# Autodesk Inventor assembly: LegAssembly
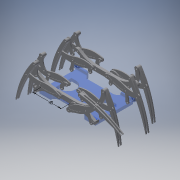
[picture p0: Inventor's stored thumbnail of the model, 180x180]
Saved by Autodesk Inventor 2017.2 (Build 212233000, 233)
## iProperties
Created: 2016-08-27
Part Number: LegAssembly
Document SubType Name: Assembly
Designer: Nic
Author: Nic
## Documents named in this file (8)
- C:\Users\Nic\Documents\TermiteBeest\LegAssembly.iam
- C:\Users\Nic\Documents\TermiteBeest\legFrame.ipt
- C:\Users\Nic\Documents\TermiteBeest\linkageC.ipt
- C:\Users\Nic\Documents\TermiteBeest\legB.ipt
- C:\Users\Nic\Documents\TermiteBeest\linkageB.ipt
- C:\Users\Nic\Documents\TermiteBeest\legA.ipt
- C:\Users\Nic\Documents\TermiteBeest\linkageA.ipt
- C:\Users\Nic\Documents\TermiteBeest\baseplate.ipt
## Components (43 placed, 7 different names)
1. legFrame:1 — Insert:1, Insert:3, Insert:4, Insert:5, Insert:6, Insert:7, Insert:8, Insert:9, Insert:10, Insert:11, Insert:12, Insert:13, Insert:14, Insert:15, Insert:61
2. legB:1 — Insert:16, Insert:17, Insert:18
3. linkageB:1 — Insert:3, Insert:4, Insert:16
4. legA:1 — Insert:17, Insert:19
5. linkageA:1 — Insert:5, Insert:19
6. linkageC:1 — Insert:6, Insert:18
7. linkageC:2 — Insert:8, Insert:20
8. linkageB:2 — Insert:7, Insert:21
9. linkageA:2 — Insert:9, Insert:22
10. legB:2 — Insert:20, Insert:21, Insert:23
11. legA:2 — Insert:22, Insert:23
12. linkageC:3 — Insert:10, Insert:24
13. linkageA:3 — Insert:11, Insert:25
14. linkageB:3 — Insert:12, Insert:26
15. legA:3 — Insert:25, Insert:27
16. legB:3 — Insert:24, Insert:26, Insert:27
17. linkageB:4 — Insert:13, Insert:28
18. linkageA:4 — Insert:15, Insert:29
19. linkageC:4 — Insert:14, Insert:30
20. legA:4 — Insert:29, Insert:31
21. legB:4 — Insert:28, Insert:30, Insert:31
22. baseplate:1 — Insert:1, Insert:32, Insert:61, Insert:62
23. linkageC:5 — Insert:34, Insert:35
24. linkageC:6 — Insert:36, Insert:37
25. legFrame:2 — Insert:32, Insert:33, Insert:34, Insert:36, Insert:38, Insert:39, Insert:40, Insert:41, Insert:42, Insert:43, Insert:44, Insert:45, Insert:53, Insert:62
26. linkageA:6 — Insert:38, Insert:46
27. linkageA:7 — Insert:39, Insert:47
28. legA:5 — Insert:47, Insert:48
29. legA:6 — Insert:46, Insert:49
30. legB:5 — Insert:35, Insert:48, Insert:50
31. legB:6 — Insert:37, Insert:49, Insert:51
32. linkageB:5 — Insert:40, Insert:50
33. linkageB:6 — Insert:41, Insert:51
34. linkageC:7 — Insert:42, Insert:52
35. linkageC:8 — Insert:53, Insert:54
36. linkageB:7 — Insert:33, Insert:55
37. linkageB:8 — Insert:45, Insert:56
38. linkageA:8 — Insert:43, Insert:57
39. linkageA:9 — Insert:44, Insert:58
40. legA:7 — Insert:57, Insert:59
41. legA:8 — Insert:58, Insert:60
42. legB:7 — Insert:54, Insert:55, Insert:59
43. legB:8 — Insert:52, Insert:56, Insert:60
## Relationships (61: Insert 61)
- Insert:1: legFrame:1 ↔ baseplate:1
- Insert:3 (1.5 mm): legFrame:1 ↔ linkageB:1
- Insert:4 (1.5 mm): legFrame:1 ↔ linkageB:1
- Insert:5: legFrame:1 ↔ linkageA:1
- Insert:6: legFrame:1 ↔ linkageC:1
- Insert:7 (1.5 mm): legFrame:1 ↔ linkageB:2
- Insert:8: legFrame:1 ↔ linkageC:2
- Insert:9: legFrame:1 ↔ linkageA:2
- Insert:10 (7 mm): legFrame:1 ↔ linkageC:3
- Insert:11 (7 mm): legFrame:1 ↔ linkageA:3
- Insert:12 (8.5 mm): legFrame:1 ↔ linkageB:3
- Insert:13 (8.5 mm): legFrame:1 ↔ linkageB:4
- Insert:14 (7 mm): legFrame:1 ↔ linkageC:4
- Insert:15 (7 mm): legFrame:1 ↔ linkageA:4
- Insert:16: legB:1 ↔ linkageB:1
- Insert:17: legB:1 ↔ legA:1
- Insert:18 (1.5 mm): legB:1 ↔ linkageC:1
- Insert:19: legA:1 ↔ linkageA:1
- Insert:20 (1.5 mm): linkageC:2 ↔ legB:2
- Insert:21: linkageB:2 ↔ legB:2
- Insert:22: linkageA:2 ↔ legA:2
- Insert:23: legB:2 ↔ legA:2
- Insert:24 (1.5 mm): linkageC:3 ↔ legB:3
- Insert:25: linkageA:3 ↔ legA:3
- Insert:26: linkageB:3 ↔ legB:3
- Insert:27: legA:3 ↔ legB:3
- Insert:28: linkageB:4 ↔ legB:4
- Insert:29: linkageA:4 ↔ legA:4
- Insert:30 (1.5 mm): linkageC:4 ↔ legB:4
- Insert:31: legA:4 ↔ legB:4
- Insert:32: baseplate:1 ↔ legFrame:2
- Insert:33 (8.5 mm): legFrame:2 ↔ linkageB:7
- Insert:34: linkageC:5 ↔ legFrame:2
- Insert:35 (1.5 mm): linkageC:5 ↔ legB:5
- Insert:36: linkageC:6 ↔ legFrame:2
- Insert:37 (1.5 mm): linkageC:6 ↔ legB:6
- Insert:38: legFrame:2 ↔ linkageA:6
- Insert:39: legFrame:2 ↔ linkageA:7
- Insert:40 (1.5 mm): legFrame:2 ↔ linkageB:5
- Insert:41 (1.5 mm): legFrame:2 ↔ linkageB:6
- Insert:42 (7 mm): legFrame:2 ↔ linkageC:7
- Insert:43 (7 mm): legFrame:2 ↔ linkageA:8
- Insert:44 (7 mm): legFrame:2 ↔ linkageA:9
- Insert:45 (8.5 mm): legFrame:2 ↔ linkageB:8
- Insert:46: linkageA:6 ↔ legA:6
- Insert:47: linkageA:7 ↔ legA:5
- Insert:48: legA:5 ↔ legB:5
- Insert:49: legA:6 ↔ legB:6
- Insert:50: legB:5 ↔ linkageB:5
- Insert:51: legB:6 ↔ linkageB:6
- Insert:52 (1.5 mm): linkageC:7 ↔ legB:8
- Insert:53 (7 mm): legFrame:2 ↔ linkageC:8
- Insert:54 (1.5 mm): linkageC:8 ↔ legB:7
- Insert:55: linkageB:7 ↔ legB:7
- Insert:56: linkageB:8 ↔ legB:8
- Insert:57: linkageA:8 ↔ legA:7
- Insert:58: linkageA:9 ↔ legA:8
- Insert:59: legA:7 ↔ legB:7
- Insert:60: legA:8 ↔ legB:8
- Insert:61: legFrame:1 ↔ baseplate:1
- Insert:62: baseplate:1 ↔ legFrame:2
